# Autodesk Inventor assembly: SSRC215
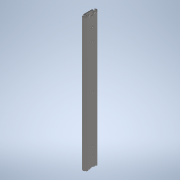
[picture p0: Inventor's stored thumbnail of the model, 180x180]
Saved by Autodesk Inventor 2022 (Build 260153000, 153)
## iProperties
Category: PARTsolutions
Company: MISUMI
Part Number: SSRC215
Catalog Web Link: www.cadenas.de
Description: SSRC2-Slide Rails - Load Rating: 137N ~ 177N/2 pcs - Light Load / Compact - Stainless Steel - Tow-Step
Vendor: MISUMI
Document SubType Name: Assembly
Designer: partserver
Manufacturer: MISUMI
Mass: 5.30611 g
Surface Area: 131.668 cm^2
Volume: 5.30611 cm^3
Density: 1 g/cm^3
PSOL_IDENT_0: {$CADENAS_DATA\23d-libs\misumi\metric\07_slide_rails\ssrc2_asmtab.prj},167 {VTYP=3D},{STYP=ASSTAB},{
PSOL_IDENT_1: NB=SSRC215},{LINA=SSRC215},{NN=SSRC2},{DATE=09.09.2019 09:02:44},{GEOMDATE=30.06.2015 02:01:53},{VER
PSOL_IDENT_2: SION=},{LINEID=30},{WBVAR=},{WBNUMERIC=}  {NB=SSRC215},{LINA=SSRC215},{KT=DUMMY},{PN=SSRC215},{TYPE=
PSOL_IDENT_3: SSRC2},{NO=15},{L=150},{S=94.5},{A=63},{B=126},{C=63},{D=126},{E=102},{F=98},{PPATH=ssrc2/ssrc2_asmt
PSOL_IDENT_4: pl.prj}
NB: SSRC215
NN: SSRC2
NT: Slide Rails - Load Rating: 137N ~ 177N/2 pcs - Light Load / Compact - Stainless Steel - Tow-Step
NBSYN: $PN.
LINA: SSRC215
CATALOG: Misumi
PN: SSRC215
NO: 15
L: 150
S: 94.5
A: 63
B: 126
C: 63
D: 126
E: 102
F: 98
SUPPLIER: MISUMI
ARTICLENO: SSRC215
BOMINFO: SSRC215
CREATOR: CADENAS GmbH
Title: SSRC215
Author: Cadenas PARTsolutions
Comments: Slide Rails - Load Rating: 137N ~ 177N/2 pcs - Light Load / Compact - Stainless Steel - Tow-Step
## Documents named in this file (4)
- C:\Users\satot\Documents\GrabCAD\NHK2022\BasicParts\SlideRail\SlideRail_94.5\SSRC215.iam
- C:\Users\satot\Documents\GrabCAD\NHK2022\BasicParts\SlideRail\SlideRail_94.5\SSRC215_or.ipt
- C:\Users\satot\Documents\GrabCAD\NHK2022\BasicParts\SlideRail\SlideRail_94.5\SSRC215_re.ipt
- C:\Users\satot\Documents\GrabCAD\NHK2022\BasicParts\SlideRail\SlideRail_94.5\SSRC215_ir.ipt
## Components (3 placed, 3 different names)
1. SSRC215_or:1 — to_retainer_Z@1 <-> to_outer_rail_Z@2, to_retainer_YZ@1 <-> to_outer_rail_YZ@2, スライダ:1
2. SSRC215_re:1 — to_retainer_Z@1 <-> to_outer_rail_Z@2, to_retainer_YZ@1 <-> to_outer_rail_YZ@2, to_inner_rail_Z@2 <-> to_retainer_Z@3, to_inner_rail_YZ@2 <-> to_retainer_YZ@3
3. SSRC215_ir:1 — to_inner_rail_Z@2 <-> to_retainer_Z@3, to_inner_rail_YZ@2 <-> to_retainer_YZ@3, スライダ:1
## Relationships (5: Mate 2, Angle 2, TranslationJoint 1)
- to_retainer_Z@1 <-> to_outer_rail_Z@2 [Mate]: SSRC215_or:1 ↔ SSRC215_re:1
- to_retainer_YZ@1 <-> to_outer_rail_YZ@2 [Angle] (0 deg): SSRC215_or:1 ↔ SSRC215_re:1
- to_inner_rail_Z@2 <-> to_retainer_Z@3 [Mate]: SSRC215_re:1 ↔ SSRC215_ir:1
- to_inner_rail_YZ@2 <-> to_retainer_YZ@3 [Angle] (180 deg): SSRC215_re:1 ↔ SSRC215_ir:1
- スライダ:1 [TranslationJoint] (4.4 mm): SSRC215_or:1 ↔ SSRC215_ir:1
